# Autodesk Inventor assembly: board_shape_test
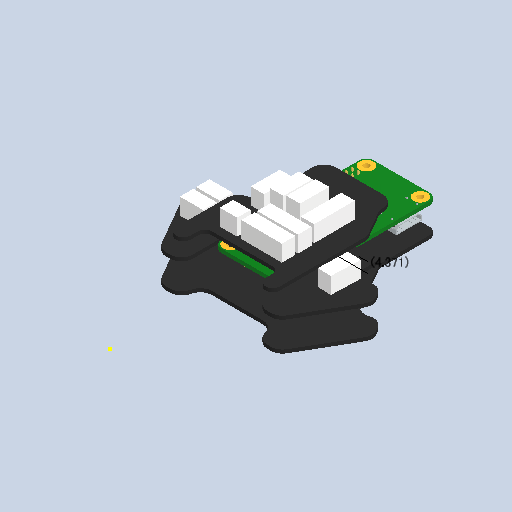
[picture p0: Inventor's stored thumbnail of the model, 512x512]
Saved by Autodesk Inventor 2024.1 (Build 281209000, 209)
## iProperties
Created: 2025-04-11
Part Number: board_shape_test
Document SubType Name: Assembly
Designer: hibik
Author: hibik
## Documents named in this file (10)
- C:\Users\hibik\Documents\Robomech\RESCUE\ORCA\hard\board\CORE\board_shape_test.iam
- C:\Users\hibik\Documents\Robomech\RESCUE\ORCA\hard\board\CORE\CORE_outline.ipt
- C:\Users\hibik\Documents\Robomech\RESCUE\ORCA\hard\board\Raspberry_PI_Zero_W.iam
- C:\Users\hibik\Documents\Robomech\RESCUE\ORCA\hard\board\CORE\CORE_hat_outline.ipt
- C:\Users\hibik\Documents\Robomech\RESCUE\ORCA\hard\board\CORE\xh\6.ipt
- C:\Users\hibik\Documents\Robomech\RESCUE\ORCA\hard\board\CORE\xh\4.ipt
- C:\Users\hibik\Documents\Robomech\RESCUE\ORCA\hard\board\CORE\xh\2.ipt
- C:\Users\hibik\Documents\Robomech\RESCUE\ORCA\hard\board\CORE\xh\3.ipt
- C:\Users\hibik\Documents\Robomech\RESCUE\ORCA\hard\board\CORE\CORE_hat_upper_outline.ipt
- C:\Users\hibik\Documents\Robomech\RESCUE\ORCA\hard\board\CORE\CORE_hat_right.ipt
## Components (15 placed, 9 different names)
1. CORE_outline:1 — メイト:1, フラッシュ:1, フラッシュ:2, メイト:2, フラッシュ:3, フラッシュ:4, フラッシュ:13, フラッシュ:14
2. Raspberry_PI_Zero_W:1 [sub-assembly] — メイト:1, フラッシュ:1, フラッシュ:2
3. CORE_hat_outline:1 — メイト:2, フラッシュ:3, フラッシュ:4, メイト:5, フラッシュ:15, フラッシュ:16, フラッシュ:17
4. CORE_hat_upper_outline:1 — メイト:5, フラッシュ:13, フラッシュ:14, メイト:7, メイト:8, メイト:9, メイト:10, メイト:13, メイト:14
5. 6:4 — メイト:7
6. 6:5 — メイト:10
7. 6:6 — メイト:13
8. 2:2 — メイト:8, メイト:9
9. 3:3 — メイト:12
10. 4:3
11. 4:4 — メイト:14
12. 3:4 — メイト:11
13. CORE_hat_right:1 — フラッシュ:15, フラッシュ:16, フラッシュ:17, メイト:11, メイト:12
14. 4:5
15. 4:6
## Relationships (20: Mate 11, Flush 9)
- メイト:1 [Mate] (11 mm): CORE_outline:1 ↔ Raspberry_PI_Zero_W:1
- フラッシュ:1 [Flush]: CORE_outline:1 ↔ Raspberry_PI_Zero_W:1
- フラッシュ:2 [Flush]: CORE_outline:1 ↔ Raspberry_PI_Zero_W:1
- メイト:2 [Mate] (11 mm): CORE_outline:1 ↔ CORE_hat_outline:1
- フラッシュ:3 [Flush]: CORE_outline:1 ↔ CORE_hat_outline:1
- フラッシュ:4 [Flush]: CORE_outline:1 ↔ CORE_hat_outline:1
- メイト:5 [Mate] (6 mm): CORE_hat_outline:1 ↔ CORE_hat_upper_outline:1
- フラッシュ:13 [Flush]: CORE_outline:1 ↔ CORE_hat_upper_outline:1
- フラッシュ:14 [Flush]: CORE_outline:1 ↔ CORE_hat_upper_outline:1
- メイト:7 [Mate]: CORE_hat_upper_outline:1 ↔ 6:4
- メイト:8 [Mate]: CORE_hat_upper_outline:1 ↔ 2:2
- メイト:9 [Mate]: CORE_hat_upper_outline:1 ↔ 2:2
- メイト:10 [Mate]: CORE_hat_upper_outline:1 ↔ 6:5
- フラッシュ:15 [Flush]: CORE_hat_outline:1 ↔ CORE_hat_right:1
- フラッシュ:16 [Flush]: CORE_hat_outline:1 ↔ CORE_hat_right:1
- フラッシュ:17 [Flush]: CORE_hat_outline:1 ↔ CORE_hat_right:1
- メイト:11 [Mate]: 3:4 ↔ CORE_hat_right:1
- メイト:12 [Mate]: 3:3 ↔ CORE_hat_right:1
- メイト:13 [Mate]: CORE_hat_upper_outline:1 ↔ 6:6
- メイト:14 [Mate]: CORE_hat_upper_outline:1 ↔ 4:4
